# Autodesk Inventor assembly: lock
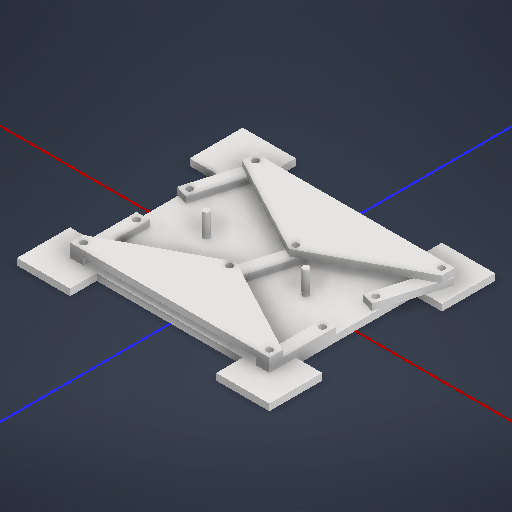
[picture p0: Inventor's stored thumbnail of the model, 512x512]
Saved by Autodesk Inventor 2025.4 (Build 294407000, 407)
## iProperties
Created: 2026-09-12
Part Number: lock
Document SubType Name: Assembly
Designer: User
Author: User
## Documents named in this file (4)
- G:\projects\secondary\computer_mechanical\gates\lock\lock.iam
- G:\projects\secondary\computer_mechanical\gates\lock\link.ipt
- G:\projects\secondary\computer_mechanical\gates\lock\bar.ipt
- G:\projects\secondary\computer_mechanical\gates\lock\base.ipt
## Components (8 placed, 3 different names)
1. link:1 — Cylindrical:6, Cylindrical:10, Mate:7
2. bar:1 — Cylindrical:7, Cylindrical:9, Cylindrical:10, Mate:4, Mate:9
3. link:2 — Cylindrical:12, Cylindrical:13, Mate:6
4. link:3 — Cylindrical:1, Cylindrical:11, Mate:5
5. link:4 — Cylindrical:5, Cylindrical:9, Mate:3, Mate:4
6. base:1 — Cylindrical:1, Cylindrical:5, Cylindrical:6, Mate:3, Cylindrical:13, Mate:5, Mate:6, Mate:7
7. bar:2 — Cylindrical:8, Cylindrical:11, Cylindrical:12, Mate:8
8. link:5 — Cylindrical:7, Cylindrical:8, Mate:8, Mate:9
## Relationships (17: CylindricalJoint 10, Mate 7)
- Cylindrical:1: link:3 ↔ base:1
- Cylindrical:5: link:4 ↔ base:1
- Cylindrical:6: link:1 ↔ base:1
- Cylindrical:7: bar:1 ↔ link:5
- Cylindrical:8: bar:2 ↔ link:5
- Cylindrical:9: bar:1 ↔ link:4
- Cylindrical:10: link:1 ↔ bar:1
- Mate:3: link:4 ↔ base:1
- Mate:4: bar:1 ↔ link:4
- Cylindrical:11: link:3 ↔ bar:2
- Cylindrical:12: link:2 ↔ bar:2
- Cylindrical:13: link:2 ↔ base:1
- Mate:5: link:3 ↔ base:1
- Mate:6: link:2 ↔ base:1
- Mate:7: link:1 ↔ base:1
- Mate:8: bar:2 ↔ link:5
- Mate:9: bar:1 ↔ link:5
